# Autodesk Inventor assembly: Gestell
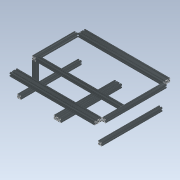
[picture p0: Inventor's stored thumbnail of the model, 180x180]
Saved by Autodesk Inventor 2022.2 (Build 262287000, 287)
## iProperties
Created: 2021-11-30
Part Number: Gestell
Document SubType Name: Assembly
Designer: Fabijan_Sven
Author: Fabijan_Sven
## Documents named in this file (9)
- H:\Sync-Folder\Sync\Hivemind\1-MCI-Unterlagen\Master\Semester 3\Projekt 2\011_Kartesischer_Roboter_Modul\07-CAD Files\01-Gestell_u_Kabelfuehrung\Gestell.iam
- H:\Sync-Folder\Sync\Hivemind\1-MCI-Unterlagen\Master\Semester 3\Projekt 2\011_Kartesischer_Roboter_Modul\07-CAD Files\01-Gestell_u_Kabelfuehrung\Profil_40x20_460.ipt
- H:\Sync-Folder\Sync\Hivemind\1-MCI-Unterlagen\Master\Semester 3\Projekt 2\011_Kartesischer_Roboter_Modul\07-CAD Files\01-Gestell_u_Kabelfuehrung\Profil_20x20_330.ipt
- H:\Sync-Folder\Sync\Hivemind\1-MCI-Unterlagen\Master\Semester 3\Projekt 2\011_Kartesischer_Roboter_Modul\07-CAD Files\01-Gestell_u_Kabelfuehrung\Profil_20x20_460.ipt
- H:\Sync-Folder\Sync\Hivemind\1-MCI-Unterlagen\Master\Semester 3\Projekt 2\011_Kartesischer_Roboter_Modul\07-CAD Files\01-Gestell_u_Kabelfuehrung\Profil_20x20_230.ipt
- H:\Sync-Folder\Sync\Hivemind\1-MCI-Unterlagen\Master\Semester 3\Projekt 2\011_Kartesischer_Roboter_Modul\07-CAD Files\01-Gestell_u_Kabelfuehrung\Profil_20x20_100.ipt
- H:\Sync-Folder\Sync\Hivemind\1-MCI-Unterlagen\Master\Semester 3\Projekt 2\011_Kartesischer_Roboter_Modul\07-CAD Files\01-Gestell_u_Kabelfuehrung\Profil_40x20_500.ipt
- H:\Sync-Folder\Sync\Hivemind\1-MCI-Unterlagen\Master\Semester 3\Projekt 2\011_Kartesischer_Roboter_Modul\07-CAD Files\01-Gestell_u_Kabelfuehrung\Profil_20x20_500.ipt
- H:\Sync-Folder\Sync\Hivemind\1-MCI-Unterlagen\Master\Semester 3\Projekt 2\011_Kartesischer_Roboter_Modul\07-CAD Files\01-Gestell_u_Kabelfuehrung\Profil_20x20_370.ipt
## Components (22 placed, 8 different names)
1. Profil_40x20_425:1
2. Profil_40x20_425:2
3. Profil_40x20_425:3
4. Profil_40x20_425:4
5. Profil_40x20_460:5
6. Profil_40x20_460:6
7. Profil_40x20_460:3 — Mate:21
8. Profil_40x20_460:4
9. Profil_20x20_500:1
10. Profil_20x20_500:2
11. Profil_20x20_460:1 — Mate:21
12. Profil_20x20_370:1
13. Profil_20x20_370:2
14. Profil_20x20_330:12
15. Profil_20x20_330:13
16. Profil_20x20_330:3 — Mate:15
17. Profil_20x20_330:10
18. Profil_20x20_330:11
19. Profil_20x20_330:4 — Mate:15
20. Profil_20x20_330:6
21. Profil_20x20_230:7 — Flush:34
22. Profil_20x20_100:1 — Flush:34
## Relationships (61: Flush 36, Mate 25)
- [Mate]: Profil_40x20_460:5 ↔ Profil_20x20_330:4
- [Flush]: Profil_40x20_460:5 ↔ Profil_20x20_330:4
- [Mate]: Profil_40x20_460:5 ↔ Profil_20x20_330:3
- [Flush]: Profil_40x20_460:5 ↔ Profil_20x20_330:3
- [Mate] (2 mm): Profil_20x20_330:13 ↔ Profil_20x20_330:4
- Mate:15 (200 mm): Profil_20x20_330:3 ↔ Profil_20x20_330:4
- [Mate]: Profil_40x20_425:1 ↔ Profil_40x20_460:3
- [Flush]: Profil_40x20_425:1 ↔ Profil_40x20_460:3
- [Flush] (120 mm): Profil_40x20_460:6 ↔ Profil_40x20_460:3
- [Mate]: Profil_40x20_425:2 ↔ Profil_20x20_330:6
- [Flush]: Profil_40x20_425:2 ↔ Profil_20x20_330:6
- [Flush] (120 mm): Profil_20x20_330:13 ↔ Profil_20x20_330:6
- [Mate]: Profil_40x20_425:4 ↔ Profil_40x20_460:4
- [Flush]: Profil_40x20_425:4 ↔ Profil_40x20_460:4
- [Flush] (120 mm): Profil_40x20_460:5 ↔ Profil_40x20_460:4
- Mate:21 (100 mm): Profil_40x20_460:3 ↔ Profil_20x20_460:1
- [Mate]: Profil_40x20_425:3 ↔ Profil_20x20_230:7
- [Flush] (120 mm): Profil_20x20_330:12 ↔ Profil_20x20_230:7
- [Flush]: Profil_40x20_425:3 ↔ Profil_20x20_230:7
- [Mate]: Profil_20x20_330:12 ↔ Profil_20x20_100:1
- [Flush]: Profil_20x20_330:12 ↔ Profil_20x20_100:1
- Flush:34: Profil_20x20_230:7 ↔ Profil_20x20_100:1
- [Mate]: Profil_40x20_460:6 ↔ Profil_20x20_330:11
- [Flush]: Profil_40x20_460:6 ↔ Profil_20x20_330:11
- [Mate]: Profil_40x20_460:6 ↔ Profil_20x20_330:10
- [Flush]: Profil_40x20_460:6 ↔ Profil_20x20_330:10
- [Mate]: Profil_20x20_330:12 ↔ Profil_20x20_330:10
- [Mate] (198 mm): Profil_20x20_330:12 ↔ Profil_20x20_330:11
- [Mate]: Profil_40x20_425:1 ↔ Profil_20x20_500:1
- [Flush]: Profil_40x20_425:1 ↔ Profil_20x20_500:1
- [Flush]: Profil_40x20_425:1 ↔ Profil_20x20_500:1
- [Mate]: Profil_40x20_425:2 ↔ Profil_20x20_500:1
- [Flush]: Profil_40x20_425:2 ↔ Profil_20x20_500:1
- [Flush]: Profil_40x20_425:2 ↔ Profil_20x20_500:1
- [Mate]: Profil_20x20_500:1 ↔ Profil_20x20_370:1
- [Flush]: Profil_20x20_500:1 ↔ Profil_20x20_370:1
- [Flush]: Profil_20x20_500:1 ↔ Profil_20x20_370:1
- [Mate]: Profil_20x20_500:1 ↔ Profil_20x20_370:2
- [Flush]: Profil_20x20_500:1 ↔ Profil_20x20_370:2
- [Flush]: Profil_20x20_500:1 ↔ Profil_20x20_370:2
- [Flush]: Profil_20x20_500:2 ↔ Profil_20x20_370:2
- [Flush]: Profil_20x20_500:2 ↔ Profil_20x20_370:2
- [Mate]: Profil_20x20_500:2 ↔ Profil_20x20_370:2
- [Mate]: Profil_40x20_425:4 ↔ Profil_20x20_500:2
- [Flush]: Profil_40x20_425:4 ↔ Profil_20x20_500:2
- [Flush]: Profil_40x20_425:4 ↔ Profil_20x20_500:2
- [Mate]: Profil_40x20_425:3 ↔ Profil_20x20_370:1
- [Flush]: Profil_40x20_425:3 ↔ Profil_20x20_500:2
- [Flush]: Profil_40x20_425:3 ↔ Profil_20x20_500:2
- [Mate]: Profil_40x20_425:4 ↔ Profil_40x20_460:5
- [Flush]: Profil_40x20_425:4 ↔ Profil_40x20_460:5
- [Flush]: Profil_40x20_425:4 ↔ Profil_40x20_460:5
- [Mate]: Profil_40x20_425:2 ↔ Profil_40x20_460:6
- [Flush]: Profil_40x20_425:2 ↔ Profil_40x20_460:6
- [Flush]: Profil_40x20_425:2 ↔ Profil_40x20_460:6
- [Mate]: Profil_40x20_425:1 ↔ Profil_20x20_330:12
- [Flush]: Profil_40x20_425:1 ↔ Profil_20x20_330:12
- [Flush]: Profil_40x20_425:1 ↔ Profil_20x20_330:12
- [Mate]: Profil_40x20_425:2 ↔ Profil_20x20_330:13
- [Flush]: Profil_40x20_425:2 ↔ Profil_20x20_330:13
- [Flush]: Profil_40x20_425:2 ↔ Profil_20x20_330:13
## Named parameters: RingHeight = 120 mm, d0_d1 = 0 mm, d1_d2 = 0 mm, d2_d3 = 0 mm, d3_d4 = 0 mm, d4_d5 = 0 mm, d5_d6 = 0 mm, d6_d7 = 0 mm, d7_d8 = 0 mm, d8_d9 = 0 mm, d9_d10 = 0 mm, d10_d11 = 0 mm, d11_d12 = 0 mm, d12_d13 = 0 mm, d13_d14 = 0 mm, d14_d15 = 0 mm, d15_d16 = 0 mm, d16_d17 = 0 mm, d17_d18 = 0 mm, d18_d19 = 0 mm, d19_d20 = 0 mm, d20_d21 = 0 mm, d21_d22 = 0 mm, d22_d23 = 0 mm, d23_d24 = 0 mm, d24_d25 = 0 mm, d25_d26 = 0 mm, d26_d27 = 0 mm, d27_d29 = 0 mm, d28_d30 = 0 mm, d29_d31 = 0 mm, d30_d32 = 0 mm
